# Autodesk Inventor assembly: Нога левая в сборе
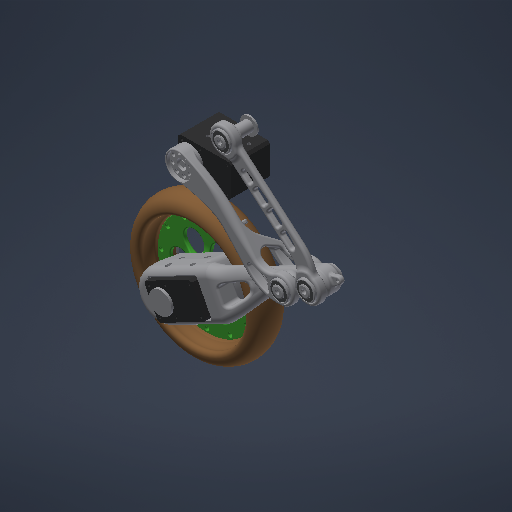
[picture p0: Inventor's stored thumbnail of the model, 512x512]
Saved by Autodesk Inventor 2025 (Build 290162010, 162A)
## iProperties
Created: 2024-06-21
Part Number: Нога левая в сборе
Document SubType Name: Assembly
Designer: Edward_Higgins
Author: Edward_Higgins
## Documents named in this file (17)
- D:\Users\Edward_Higgins\Desktop\ZAVOD\Робот Сколково\Нога левая в сборе.iam
- D:\Users\Edward_Higgins\Desktop\ZAVOD\Робот Сколково\Тяга передняя.ipt
- D:\Users\Edward_Higgins\Desktop\ZAVOD\Робот Сколково\DYNAMIXEL XM430-W350.ipt
- D:\Users\Edward_Higgins\Desktop\ZAVOD\Робот Сколково\Корпус ноги.ipt
- D:\Users\Edward_Higgins\Desktop\ZAVOD\Робот Сколково\Тяга задняя 2.ipt
- D:\Users\Edward_Higgins\Desktop\ZAVOD\Робот Сколково\Голень в сборе.iam
- D:\Users\Edward_Higgins\Desktop\ZAVOD\Робот Сколково\Подшипник.ipt
- D:\Users\Edward_Higgins\Desktop\ZAVOD\Робот Сколково\Стопорная шайба.ipt
- D:\Users\Edward_Higgins\Desktop\ZAVOD\Робот Сколково\Шайба.ipt
- D:\Users\Edward_Higgins\Desktop\ZAVOD\Робот Сколково\Ось односторонняя.ipt
- D:\Users\Edward_Higgins\Desktop\ZAVOD\Робот Сколково\Колесо 2 в сборе.iam
- D:\Users\Edward_Higgins\Desktop\ZAVOD\Робот Сколково\Нога левая в сборе\AIP\FEA\ew5x1yt5s.fins
- D:\Users\Edward_Higgins\Desktop\ZAVOD\Робот Сколково\Нога левая в сборе\AIP\FEA\ew5x1yt5s.fsat
- D:\Users\Edward_Higgins\Desktop\ZAVOD\Робот Сколково\Нога левая в сборе\AIP\FEA\ew5x1yt5s.ftes
- D:\Users\Edward_Higgins\Desktop\ZAVOD\Робот Сколково\Нога левая в сборе\AIP\FEA\ew5x1yt5s.fwiz
- D:\Users\Edward_Higgins\Desktop\ZAVOD\Робот Сколково\Нога левая в сборе\AIP\FEA\ew5x1yt6o.fmsh
- D:\Users\Edward_Higgins\Desktop\ZAVOD\Робот Сколково\Нога левая в сборе\AIP\FEA\ew5x1yt6p.fres
## Components (10 placed, 10 different names)
1. Тяга передняя:1 — Совмещение:21, Совмещение:82, Совмещение:84, Совмещение:85
2. DYNAMIXEL XM430-W350:2 — Совмещение:21, Совмещение:30, Угол:1, Совмещение:83, Совмещение:84
3. Корпус ноги:1 — Совмещение:14, Совмещение:15, Совмещение:30, Угол:1, Совмещение:83, Совмещение:95, Совмещение:98, Совмещение:103
4. Голень в сборе:1 [sub-assembly] — Совмещение:82, Совмещение:85, Совмещение:99, Совмещение:100, Совмещение:104, Совмещение:105
5. Подшипник:1 — Совмещение:102
6. Стопорная шайба:1
7. Шайба:1 — Совмещение:96, Совмещение:103
8. Ось односторонняя:1 — Совмещение:95, Совмещение:96, Совмещение:98
9. Колесо 2 в сборе:1 [sub-assembly] — Совмещение:99, Совмещение:100
10. Тяга задняя 2:3 — Совмещение:102, Совмещение:104, Совмещение:105
## Relationships (23: Mate 22, Angle 1)
- Совмещение:14 [Mate]: Корпус ноги:1
- Совмещение:15 [Mate]: Корпус ноги:1
- Совмещение:21 [Mate]: Тяга передняя:1 ↔ DYNAMIXEL XM430-W350:2
- Совмещение:30 [Mate]: DYNAMIXEL XM430-W350:2 ↔ Корпус ноги:1
- Угол:1 [Angle] (0 deg): DYNAMIXEL XM430-W350:2 ↔ Корпус ноги:1
- Совмещение:82 [Mate]: Тяга передняя:1 ↔ Голень в сборе:1
- Совмещение:83 [Mate]: DYNAMIXEL XM430-W350:2 ↔ Корпус ноги:1
- Совмещение:84 [Mate]: Тяга передняя:1 ↔ DYNAMIXEL XM430-W350:2
- Совмещение:85 [Mate]: Тяга передняя:1 ↔ Голень в сборе:1
- [Mate]: Подшипник:1 ↔ Стопорная шайба:1
- [Mate]: Подшипник:1 ↔ Стопорная шайба:1
- [Mate]: Подшипник:1 ↔ Ось односторонняя:1
- [Mate]: Подшипник:1 ↔ Ось односторонняя:1
- [Mate]: Шайба:1 ↔ Ось односторонняя:1
- Совмещение:95 [Mate]: Корпус ноги:1 ↔ Ось односторонняя:1
- Совмещение:96 [Mate]: Шайба:1 ↔ Ось односторонняя:1
- Совмещение:98 [Mate]: Корпус ноги:1 ↔ Ось односторонняя:1
- Совмещение:99 [Mate]: Голень в сборе:1 ↔ Колесо 2 в сборе:1
- Совмещение:100 [Mate]: Голень в сборе:1 ↔ Колесо 2 в сборе:1
- Совмещение:102 [Mate]: Подшипник:1 ↔ Тяга задняя 2:3
- Совмещение:103 [Mate]: Корпус ноги:1 ↔ Шайба:1
- Совмещение:104 [Mate]: Голень в сборе:1 ↔ Тяга задняя 2:3
- Совмещение:105 [Mate]: Голень в сборе:1 ↔ Тяга задняя 2:3
## Named parameters: d26_d24 = 0 mm, d27_d25 = 0 mm, sa_0 = 5000
note: some values were not read from the file. Shown as the stored number, unit unknown: "sa_0".
